# Autodesk Inventor assembly: BodyRod-KST215MG
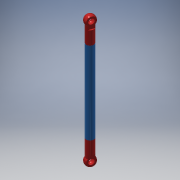
[picture p0: Inventor's stored thumbnail of the model, 180x180]
Saved by Autodesk Inventor 2018.2 (Build 222227000, 227)
## iProperties
Created: 2018-02-25
Part Number: BodyRod-KST215MG
Material: Generisch
Document SubType Name: Assembly
Designer: JochenAlt
Author: JochenAlt
## Documents named in this file (3)
- D:\Projects\Donna\CAD\Body-Rod.iam
- D:\Projects\Donna\CAD\Ball-Joint Female.ipt
- D:\Projects\Donna\CAD\Stewart-Body-Rod-Pipe.ipt
## Components (3 placed, 2 different names)
1. Ball Joint Female:1 — Passend:1, Passend:2, Passend:3, Passend:4, Winkel:1
2. Ball Joint Female:2 — Passend:5, Passend:6, Winkel:1
3. Stewart-Body-Rod-Pipe:1 — Passend:3, Passend:4, Passend:5, Passend:6
## Relationships (7: Mate 6, Angle 1)
- Passend:1 [Mate]: Ball Joint Female:1
- Passend:2 [Mate]: Ball Joint Female:1
- Passend:3 [Mate]: Ball Joint Female:1 ↔ Stewart-Body-Rod-Pipe:1
- Passend:4 [Mate]: Ball Joint Female:1 ↔ Stewart-Body-Rod-Pipe:1
- Passend:5 [Mate]: Ball Joint Female:2 ↔ Stewart-Body-Rod-Pipe:1
- Passend:6 [Mate]: Ball Joint Female:2 ↔ Stewart-Body-Rod-Pipe:1
- Winkel:1 [Angle] (0 deg): Ball Joint Female:1 ↔ Ball Joint Female:2
